# Autodesk Inventor assembly: Mechaniczny_panel_tylny_regal_V1_1
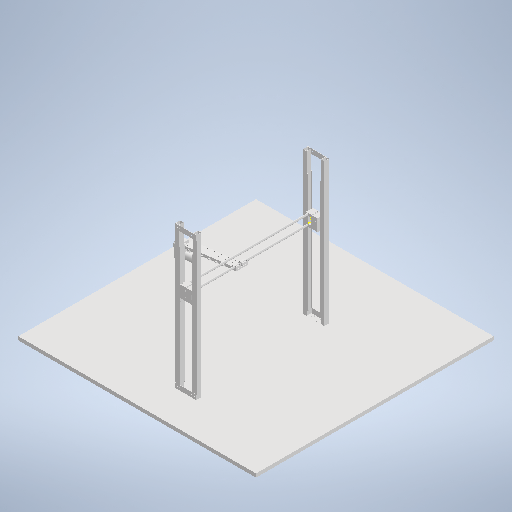
[picture p0: Inventor's stored thumbnail of the model, 512x512]
Saved by Autodesk Inventor 2025.2 (Build 292293000, 293)
## iProperties
Created: 2025-03-18
Part Number: Mechaniczny_panel_tylny_regal_V1_1
Document SubType Name: Assembly
Designer: tadek
Author: tadek
## Documents named in this file (30)
- C:\Users\tadek\Documents\Inventor_projekt_inzynierski\Mechaniczny_panel_tylny_regal_V1_1.iam
- C:\Users\tadek\Documents\Inventor_projekt_inzynierski\lacznik_plaski_180_40_2p5.ipt
- C:\Users\tadek\Documents\Inventor_projekt_inzynierski\podstawa_plyta_200_200_3.ipt
- C:\Users\tadek\Documents\Inventor_projekt_inzynierski\profil_stalowy_40_30_120_MIR.ipt
- C:\Users\tadek\Documents\Inventor_projekt_inzynierski\katownik_lacznikowy_40_40_40.ipt
- C:\Users\tadek\Documents\Inventor_projekt_inzynierski\prowadnica_profil_c.ipt
- C:\Users\tadek\Documents\Inventor_projekt_inzynierski\prowadnica_profil_c_MIR.ipt
- C:\Users\tadek\Documents\Inventor_projekt_inzynierski\lozysko.ipt
- C:\Users\tadek\Documents\Inventor_projekt_inzynierski\lozysko_MIR.ipt
- C:\Users\tadek\Documents\Inventor_projekt_inzynierski\katownik_lacznikowy_40_40_40_MIR1.ipt
- C:\Users\tadek\Documents\Inventor_projekt_inzynierski\lacznik_lozyskowy.ipt
- C:\Users\tadek\Documents\Inventor\Content Center Files\R2025\pl-PL\PEM Self-Clinching Studs FH4,FHP - Metric\FH4-M5-8.ipt
- C:\Users\tadek\Documents\Inventor_projekt_inzynierski\nakretka.ipt
- C:\Users\tadek\Documents\Inventor_projekt_inzynierski\profil_stalowy_40_30_120_MIR_MIR1.ipt
- C:\Users\tadek\Documents\Inventor_projekt_inzynierski\prowadnica_profil_c_MIR2.ipt
- C:\Users\tadek\Documents\Inventor_projekt_inzynierski\prowadnica_profil_c_MIR_MIR1.ipt
- C:\Users\tadek\Documents\Inventor_projekt_inzynierski\lozysko_MIR2.ipt
- C:\Users\tadek\Documents\Inventor_projekt_inzynierski\lozysko_MIR_MIR1.ipt
- C:\Users\tadek\Documents\Inventor_projekt_inzynierski\lacznik_lozyskowy_MIR.ipt
- C:\Users\tadek\Documents\Inventor_projekt_inzynierski\nakretka_MIR.ipt
- C:\Users\tadek\Documents\Inventor_projekt_inzynierski\Zespół1.iam
- C:\Users\tadek\Documents\Inventor_projekt_inzynierski\profil_stalowy_40_30_120_MIR_MIR1_CPY.ipt
- C:\Users\tadek\Documents\Inventor_projekt_inzynierski\profil_stalowy_40_30_120_MIR_CPY.ipt
- C:\Users\tadek\Documents\Inventor_projekt_inzynierski\katownik_lacznikowy_40_40_40_CPY.ipt
- C:\Users\tadek\Documents\Inventor_projekt_inzynierski\katownik_lacznikowy_40_40_40_MIR1_CPY.ipt
- C:\Users\tadek\Documents\Inventor_projekt_inzynierski\lacznik_plaski_180_40_2p5_CPY.ipt
- C:\Users\tadek\Documents\Inventor_projekt_inzynierski\prowadnica_profil_c_CPY.ipt
- C:\Users\tadek\Documents\Inventor_projekt_inzynierski\prowadnica_profil_c_MIR2_CPY.ipt
- C:\Users\tadek\Documents\Inventor_projekt_inzynierski\prowadnica_profil_c_MIR_CPY.ipt
- C:\Users\tadek\Documents\Inventor_projekt_inzynierski\prowadnica_profil_c_MIR_MIR1_CPY.ipt
## Components (50 placed, 29 different names)
1. Zespół1:1 [sub-assembly] — Zestawiające:103, Zestawiające:104, Zestawiające:109, Zestawiające:110, Zestawiające:112, Zestawiające:113, Zestawiające:114, Zestawiające:115, Zestawiające:116, Zestawiające:119, Zestawiające:120, Zestawiające:121, Zestawiające:195, Zestawiające:223, Zestawiające:225, Zestawiające:226, Zestawiające:227, Zestawiające:228, Zestawiające:242, Zestawiające:243
2. podstawa_plyta_200_200_3:1 — Równoległe:9, Równoległe:11, Zestawiające:22, Zestawiające:39, Zestawiające:40, Zestawiające:41, Zestawiające:42, Zestawiające:43, Zestawiające:91, Zestawiające:92, Zestawiające:187, Zestawiające:188, Zestawiające:191, Zestawiające:192, Zestawiające:193, Zestawiające:194
3. profil_stalowy_40_30_120_MIR_MIR1:1 — Zestawiające:63, Zestawiające:64, Zestawiające:65, Zestawiające:66, Zestawiające:67, Zestawiające:68, Zestawiające:74, Zestawiające:75, Zestawiające:76, Zestawiające:77, Zestawiające:93, Zestawiające:94, Zestawiające:95, Zestawiające:96, Zestawiające:123, Zestawiające:124
4. profil_stalowy_40_30_120_MIR:1 — Równoległe:6, Równoległe:8, Zestawiające:4, Zestawiające:5, Równoległe:9, Zestawiające:7, Zestawiające:9, Zestawiające:10, Zestawiające:11, Zestawiające:12, Zestawiające:13, Zestawiające:14, Zestawiające:15, Zestawiające:20, Zestawiające:21, Zestawiające:44, Zestawiające:45, Zestawiające:46, Zestawiające:47, Zestawiające:122
5. lacznik_lozyskowy:1 — Zestawiające:51, Zestawiające:53, Zestawiające:52, Zestawiające:54, Zestawiające:103, Zestawiające:109, Zestawiające:110, Zestawiające:112, Zestawiające:113
6. lacznik_lozyskowy_MIR:1 — Zestawiające:71, Zestawiające:104, Zestawiające:105, Zestawiające:106, Zestawiające:114, Zestawiające:115, Zestawiające:116, Zestawiające:119, Zestawiające:120, Zestawiające:121
7. katownik_lacznikowy_40_40_40:1 — Zestawiające:7, Równoległe:11, Zestawiające:9, Zestawiające:20, Zestawiające:21, Zestawiające:22, Zestawiające:42, Zestawiające:43, Zestawiające:44, Zestawiające:45, Zestawiające:46
8. katownik_lacznikowy_40_40_40_MIR1:1 — Zestawiające:39, Zestawiające:40, Zestawiające:41, Zestawiające:74, Zestawiające:75, Zestawiające:76, Zestawiające:77, Zestawiające:91, Zestawiające:92
9. lacznik_plaski_180_40_2p5:1 — Zestawiające:4, Zestawiające:5, Zestawiające:95, Zestawiające:96, Zestawiające:122, Zestawiające:123, Zestawiające:124
10. lacznik_plaski_180_40_2p5:2 — Zestawiające:47, Zestawiające:93, Zestawiające:94
11. prowadnica_profil_c:2 — Zestawiające:10, Zestawiające:11, Zestawiające:12, Zestawiające:16, Zestawiające:17
12. prowadnica_profil_c_MIR2:1 — Zestawiające:63, Zestawiające:64, Zestawiające:65, Zestawiające:69
13. prowadnica_profil_c_MIR:1 — Zestawiające:13, Zestawiające:14, Zestawiające:15, Zestawiające:18, Zestawiające:19
14. prowadnica_profil_c_MIR_MIR1:1 — Zestawiające:66, Zestawiające:67, Zestawiające:68, Zestawiające:70, Równoległe:15
15. PEM Śruba dwustronna samozaciskowa FH4,FHP - Metryczny FH4-M5-8:2 — Zestawiające:53, Zestawiające:54, Zestawiające:55, Zestawiające:57, Zestawiające:111
16. PEM Śruba dwustronna samozaciskowa FH4,FHP - Metryczny FH4-M5-8:1 — Zestawiające:51, Zestawiające:52, Zestawiające:56, Zestawiające:59
17. PEM Śruba dwustronna samozaciskowa FH4,FHP - Metryczny FH4-M5-8:3 — Zestawiające:86, Zestawiające:90, Zestawiające:105, Zestawiające:118
18. PEM Śruba dwustronna samozaciskowa FH4,FHP - Metryczny FH4-M5-8:4 — Zestawiające:85, Zestawiające:89, Zestawiające:106, Zestawiające:117
19. nakretka:1 — Zestawiające:59, Zestawiające:62
20. nakretka_MIR:1 — Zestawiające:72, Zestawiające:89, Zestawiające:117
21. nakretka:2 — Zestawiające:57, Zestawiające:61, Zestawiające:111
22. nakretka_MIR:2 — Zestawiające:73, Zestawiające:90, Zestawiające:118
23. lozysko:1 — Zestawiające:16, Zestawiające:17, Zestawiające:56, Zestawiające:62
24. lozysko_MIR:1 — Zestawiające:18, Zestawiające:19, Zestawiające:55, Zestawiające:61
25. lozysko_MIR2:1 — Zestawiające:69, Zestawiające:71, Zestawiające:72, Zestawiające:85
26. lozysko_MIR_MIR1:1 — Zestawiające:70, Równoległe:15, Zestawiające:73, Zestawiające:86
27. profil_stalowy_40_30_120_MIR_CPY:1 — Zestawiające:125, Zestawiające:126, Zestawiające:127, Równoległe:17, Zestawiające:128, Zestawiające:129, Zestawiające:130, Zestawiające:131, Zestawiające:132, Zestawiające:133, Zestawiające:134, Zestawiające:135, Zestawiające:136, Zestawiające:137, Zestawiające:138, Zestawiające:139, Zestawiające:140, Zestawiające:145, Równoległe:19
28. profil_stalowy_40_30_120_MIR_MIR1_CPY:1 — Zestawiające:157, Zestawiające:158, Zestawiające:159, Zestawiające:160, Zestawiające:161, Zestawiające:162, Zestawiające:163, Zestawiające:164, Zestawiające:165, Zestawiające:166, Zestawiające:167, Zestawiające:168, Zestawiające:169, Zestawiające:170, Zestawiające:171, Zestawiające:172
29. lacznik_lozyskowy:2 — Zestawiające:242, Zestawiające:243
30. lacznik_lozyskowy_MIR:2 — Zestawiające:222, Zestawiające:223, Zestawiające:225, Zestawiające:226, Zestawiające:227, Zestawiające:228
31. lacznik_plaski_180_40_2p5_CPY:2 — Zestawiające:145, Zestawiające:161, Zestawiające:162
32. lacznik_plaski_180_40_2p5_CPY:1 — Zestawiające:125, Zestawiające:126, Zestawiające:127, Zestawiające:157, Zestawiające:158, Zestawiające:159, Zestawiające:160
33. katownik_lacznikowy_40_40_40_MIR1_CPY:1 — Zestawiające:163, Zestawiające:164, Zestawiające:165, Zestawiające:166, Zestawiające:188, Zestawiające:192, Zestawiające:193, Zestawiające:194
34. katownik_lacznikowy_40_40_40_CPY:1 — Zestawiające:128, Zestawiające:129, Zestawiające:130, Zestawiające:131, Zestawiające:132, Zestawiające:133, Zestawiające:134, Zestawiające:187, Zestawiające:191
35. prowadnica_profil_c_MIR_MIR1_CPY:1 — Zestawiające:170, Zestawiające:171, Zestawiające:172, Zestawiające:245
36. prowadnica_profil_c_MIR_CPY:1 — Zestawiające:138, Zestawiające:139, Zestawiające:140
37. prowadnica_profil_c_MIR2_CPY:1 — Zestawiające:167, Zestawiające:168, Zestawiające:169
38. prowadnica_profil_c_CPY:1 — Zestawiające:135, Zestawiające:136, Zestawiające:137, Zestawiające:244
39. PEM Śruba dwustronna samozaciskowa FH4,FHP - Metryczny FH4-M5-8:12
40. PEM Śruba dwustronna samozaciskowa FH4,FHP - Metryczny FH4-M5-8:11 — Zestawiające:240, Zestawiające:241
41. PEM Śruba dwustronna samozaciskowa FH4,FHP - Metryczny FH4-M5-8:10
42. PEM Śruba dwustronna samozaciskowa FH4,FHP - Metryczny FH4-M5-8:9 — Zestawiające:222
43. nakretka:4
44. nakretka:3 — Zestawiające:241
45. nakretka_MIR:4
46. nakretka_MIR:3
47. lozysko:2 — Zestawiające:240, Zestawiające:245
48. lozysko_MIR:2
49. lozysko_MIR_MIR1:2 — Zestawiające:244
50. lozysko_MIR2:2
## Relationships (162: Mate 155, Flush 7)
- Równoległe:6 [Flush]: profil_stalowy_40_30_120_MIR:1
- Równoległe:8 [Flush] (120 mm): profil_stalowy_40_30_120_MIR:1
- Zestawiające:4 [Mate]: profil_stalowy_40_30_120_MIR:1 ↔ lacznik_plaski_180_40_2p5:1
- Zestawiające:5 [Mate]: profil_stalowy_40_30_120_MIR:1 ↔ lacznik_plaski_180_40_2p5:1
- Równoległe:9 [Flush]: podstawa_plyta_200_200_3:1 ↔ profil_stalowy_40_30_120_MIR:1
- Zestawiające:7 [Mate]: profil_stalowy_40_30_120_MIR:1 ↔ katownik_lacznikowy_40_40_40:1
- Równoległe:11 [Flush]: podstawa_plyta_200_200_3:1 ↔ katownik_lacznikowy_40_40_40:1
- Zestawiające:9 [Mate]: profil_stalowy_40_30_120_MIR:1 ↔ katownik_lacznikowy_40_40_40:1
- Zestawiające:10 [Mate]: profil_stalowy_40_30_120_MIR:1 ↔ prowadnica_profil_c:2
- Zestawiające:11 [Mate]: profil_stalowy_40_30_120_MIR:1 ↔ prowadnica_profil_c:2
- Zestawiające:12 [Mate]: profil_stalowy_40_30_120_MIR:1 ↔ prowadnica_profil_c:2
- Zestawiające:13 [Mate]: profil_stalowy_40_30_120_MIR:1 ↔ prowadnica_profil_c_MIR:1
- Zestawiające:14 [Mate]: profil_stalowy_40_30_120_MIR:1 ↔ prowadnica_profil_c_MIR:1
- Zestawiające:15 [Mate]: profil_stalowy_40_30_120_MIR:1 ↔ prowadnica_profil_c_MIR:1
- Zestawiające:16 [Mate]: prowadnica_profil_c:2 ↔ lozysko:1
- Zestawiające:17 [Mate] (8 mm): prowadnica_profil_c:2 ↔ lozysko:1
- Zestawiające:18 [Mate]: prowadnica_profil_c_MIR:1 ↔ lozysko_MIR:1
- Zestawiające:19 [Mate] (8 mm): prowadnica_profil_c_MIR:1 ↔ lozysko_MIR:1
- Zestawiające:20 [Mate]: profil_stalowy_40_30_120_MIR:1 ↔ katownik_lacznikowy_40_40_40:1
- Zestawiające:21 [Mate]: profil_stalowy_40_30_120_MIR:1 ↔ katownik_lacznikowy_40_40_40:1
- Zestawiające:22 [Mate]: podstawa_plyta_200_200_3:1 ↔ katownik_lacznikowy_40_40_40:1
- Zestawiające:39 [Mate]: podstawa_plyta_200_200_3:1 ↔ katownik_lacznikowy_40_40_40_MIR1:1
- Zestawiające:40 [Mate]: podstawa_plyta_200_200_3:1 ↔ katownik_lacznikowy_40_40_40_MIR1:1
- Zestawiające:41 [Mate]: podstawa_plyta_200_200_3:1 ↔ katownik_lacznikowy_40_40_40_MIR1:1
- Zestawiające:42 [Mate]: podstawa_plyta_200_200_3:1 ↔ katownik_lacznikowy_40_40_40:1
- Zestawiające:43 [Mate]: podstawa_plyta_200_200_3:1 ↔ katownik_lacznikowy_40_40_40:1
- Zestawiające:44 [Mate]: profil_stalowy_40_30_120_MIR:1 ↔ katownik_lacznikowy_40_40_40:1
- Zestawiające:45 [Mate]: profil_stalowy_40_30_120_MIR:1 ↔ katownik_lacznikowy_40_40_40:1
- Zestawiające:46 [Mate]: profil_stalowy_40_30_120_MIR:1 ↔ katownik_lacznikowy_40_40_40:1
- Zestawiające:47 [Mate]: profil_stalowy_40_30_120_MIR:1 ↔ lacznik_plaski_180_40_2p5:2
- Zestawiające:51 [Mate]: lacznik_lozyskowy:1 ↔ PEM Śruba dwustronna samozaciskowa FH4,FHP - Metryczny FH4-M5-8:1
- Zestawiające:53 [Mate]: lacznik_lozyskowy:1 ↔ PEM Śruba dwustronna samozaciskowa FH4,FHP - Metryczny FH4-M5-8:2
- Zestawiające:52 [Mate]: lacznik_lozyskowy:1 ↔ PEM Śruba dwustronna samozaciskowa FH4,FHP - Metryczny FH4-M5-8:1
- Zestawiające:54 [Mate]: lacznik_lozyskowy:1 ↔ PEM Śruba dwustronna samozaciskowa FH4,FHP - Metryczny FH4-M5-8:2
- Zestawiające:55 [Mate]: PEM Śruba dwustronna samozaciskowa FH4,FHP - Metryczny FH4-M5-8:2 ↔ lozysko_MIR:1
- Zestawiające:56 [Mate]: PEM Śruba dwustronna samozaciskowa FH4,FHP - Metryczny FH4-M5-8:1 ↔ lozysko:1
- Zestawiające:57 [Mate]: PEM Śruba dwustronna samozaciskowa FH4,FHP - Metryczny FH4-M5-8:2 ↔ nakretka:2
- Zestawiające:59 [Mate]: PEM Śruba dwustronna samozaciskowa FH4,FHP - Metryczny FH4-M5-8:1 ↔ nakretka:1
- Zestawiające:61 [Mate]: nakretka:2 ↔ lozysko_MIR:1
- Zestawiające:62 [Mate]: nakretka:1 ↔ lozysko:1
- Zestawiające:63 [Mate]: profil_stalowy_40_30_120_MIR_MIR1:1 ↔ prowadnica_profil_c_MIR2:1
- Zestawiające:64 [Mate]: profil_stalowy_40_30_120_MIR_MIR1:1 ↔ prowadnica_profil_c_MIR2:1
- Zestawiające:65 [Mate]: profil_stalowy_40_30_120_MIR_MIR1:1 ↔ prowadnica_profil_c_MIR2:1
- Zestawiające:66 [Mate]: profil_stalowy_40_30_120_MIR_MIR1:1 ↔ prowadnica_profil_c_MIR_MIR1:1
- Zestawiające:67 [Mate]: profil_stalowy_40_30_120_MIR_MIR1:1 ↔ prowadnica_profil_c_MIR_MIR1:1
- Zestawiające:68 [Mate]: profil_stalowy_40_30_120_MIR_MIR1:1 ↔ prowadnica_profil_c_MIR_MIR1:1
- Zestawiające:69 [Mate] (8 mm): prowadnica_profil_c_MIR2:1 ↔ lozysko_MIR2:1
- Zestawiające:70 [Mate] (8 mm): prowadnica_profil_c_MIR_MIR1:1 ↔ lozysko_MIR_MIR1:1
- Równoległe:15 [Flush]: prowadnica_profil_c_MIR_MIR1:1 ↔ lozysko_MIR_MIR1:1
- Zestawiające:71 [Mate]: lacznik_lozyskowy_MIR:1 ↔ lozysko_MIR2:1
- Zestawiające:72 [Mate]: nakretka_MIR:1 ↔ lozysko_MIR2:1
- Zestawiające:73 [Mate]: nakretka_MIR:2 ↔ lozysko_MIR_MIR1:1
- Zestawiające:74 [Mate]: profil_stalowy_40_30_120_MIR_MIR1:1 ↔ katownik_lacznikowy_40_40_40_MIR1:1
- Zestawiające:75 [Mate]: profil_stalowy_40_30_120_MIR_MIR1:1 ↔ katownik_lacznikowy_40_40_40_MIR1:1
- Zestawiające:76 [Mate]: profil_stalowy_40_30_120_MIR_MIR1:1 ↔ katownik_lacznikowy_40_40_40_MIR1:1
- Zestawiające:77 [Mate]: profil_stalowy_40_30_120_MIR_MIR1:1 ↔ katownik_lacznikowy_40_40_40_MIR1:1
- Zestawiające:85 [Mate]: PEM Śruba dwustronna samozaciskowa FH4,FHP - Metryczny FH4-M5-8:4 ↔ lozysko_MIR2:1
- Zestawiające:86 [Mate]: PEM Śruba dwustronna samozaciskowa FH4,FHP - Metryczny FH4-M5-8:3 ↔ lozysko_MIR_MIR1:1
- Zestawiające:89 [Mate]: PEM Śruba dwustronna samozaciskowa FH4,FHP - Metryczny FH4-M5-8:4 ↔ nakretka_MIR:1
- Zestawiające:90 [Mate]: PEM Śruba dwustronna samozaciskowa FH4,FHP - Metryczny FH4-M5-8:3 ↔ nakretka_MIR:2
- Zestawiające:91 [Mate]: podstawa_plyta_200_200_3:1 ↔ katownik_lacznikowy_40_40_40_MIR1:1
- Zestawiające:92 [Mate]: podstawa_plyta_200_200_3:1 ↔ katownik_lacznikowy_40_40_40_MIR1:1
- Zestawiające:93 [Mate]: profil_stalowy_40_30_120_MIR_MIR1:1 ↔ lacznik_plaski_180_40_2p5:2
- Zestawiające:94 [Mate]: profil_stalowy_40_30_120_MIR_MIR1:1 ↔ lacznik_plaski_180_40_2p5:2
- Zestawiające:95 [Mate]: profil_stalowy_40_30_120_MIR_MIR1:1 ↔ lacznik_plaski_180_40_2p5:1
- Zestawiające:96 [Mate]: profil_stalowy_40_30_120_MIR_MIR1:1 ↔ lacznik_plaski_180_40_2p5:1
- Zestawiające:103 [Mate]: Zespół1:1 ↔ lacznik_lozyskowy:1
- Zestawiające:104 [Mate]: Zespół1:1 ↔ lacznik_lozyskowy_MIR:1
- Zestawiające:105 [Mate]: lacznik_lozyskowy_MIR:1 ↔ PEM Śruba dwustronna samozaciskowa FH4,FHP - Metryczny FH4-M5-8:3
- Zestawiające:106 [Mate]: lacznik_lozyskowy_MIR:1 ↔ PEM Śruba dwustronna samozaciskowa FH4,FHP - Metryczny FH4-M5-8:4
- Zestawiające:109 [Mate]: Zespół1:1 ↔ lacznik_lozyskowy:1
- Zestawiające:110 [Mate]: Zespół1:1 ↔ lacznik_lozyskowy:1
- Zestawiające:111 [Mate]: PEM Śruba dwustronna samozaciskowa FH4,FHP - Metryczny FH4-M5-8:2 ↔ nakretka:2
- Zestawiające:112 [Mate]: Zespół1:1 ↔ lacznik_lozyskowy:1
- Zestawiające:113 [Mate]: Zespół1:1 ↔ lacznik_lozyskowy:1
- Zestawiające:114 [Mate]: Zespół1:1 ↔ lacznik_lozyskowy_MIR:1
- Zestawiające:115 [Mate]: Zespół1:1 ↔ lacznik_lozyskowy_MIR:1
- Zestawiające:116 [Mate]: Zespół1:1 ↔ lacznik_lozyskowy_MIR:1
- Zestawiające:117 [Mate]: PEM Śruba dwustronna samozaciskowa FH4,FHP - Metryczny FH4-M5-8:4 ↔ nakretka_MIR:1
- Zestawiające:118 [Mate]: PEM Śruba dwustronna samozaciskowa FH4,FHP - Metryczny FH4-M5-8:3 ↔ nakretka_MIR:2
- Zestawiające:119 [Mate]: Zespół1:1 ↔ lacznik_lozyskowy_MIR:1
- Zestawiające:120 [Mate]: Zespół1:1 ↔ lacznik_lozyskowy_MIR:1
- Zestawiające:121 [Mate]: Zespół1:1 ↔ lacznik_lozyskowy_MIR:1
- Zestawiające:122 [Mate]: profil_stalowy_40_30_120_MIR:1 ↔ lacznik_plaski_180_40_2p5:1
- Zestawiające:123 [Mate]: profil_stalowy_40_30_120_MIR_MIR1:1 ↔ lacznik_plaski_180_40_2p5:1
- Zestawiające:124 [Mate]: profil_stalowy_40_30_120_MIR_MIR1:1 ↔ lacznik_plaski_180_40_2p5:1
- Zestawiające:125 [Mate]: profil_stalowy_40_30_120_MIR_CPY:1 ↔ lacznik_plaski_180_40_2p5_CPY:1
- Zestawiające:126 [Mate]: profil_stalowy_40_30_120_MIR_CPY:1 ↔ lacznik_plaski_180_40_2p5_CPY:1
- Zestawiające:127 [Mate]: profil_stalowy_40_30_120_MIR_CPY:1 ↔ lacznik_plaski_180_40_2p5_CPY:1
- Równoległe:17 [Flush] (120 mm): profil_stalowy_40_30_120_MIR_CPY:1
- Zestawiające:128 [Mate]: profil_stalowy_40_30_120_MIR_CPY:1 ↔ katownik_lacznikowy_40_40_40_CPY:1
- Zestawiające:129 [Mate]: profil_stalowy_40_30_120_MIR_CPY:1 ↔ katownik_lacznikowy_40_40_40_CPY:1
- Zestawiające:130 [Mate]: profil_stalowy_40_30_120_MIR_CPY:1 ↔ katownik_lacznikowy_40_40_40_CPY:1
- Zestawiające:131 [Mate]: profil_stalowy_40_30_120_MIR_CPY:1 ↔ katownik_lacznikowy_40_40_40_CPY:1
- Zestawiające:132 [Mate]: profil_stalowy_40_30_120_MIR_CPY:1 ↔ katownik_lacznikowy_40_40_40_CPY:1
- Zestawiające:133 [Mate]: profil_stalowy_40_30_120_MIR_CPY:1 ↔ katownik_lacznikowy_40_40_40_CPY:1
- Zestawiające:134 [Mate]: profil_stalowy_40_30_120_MIR_CPY:1 ↔ katownik_lacznikowy_40_40_40_CPY:1
- Zestawiające:135 [Mate]: profil_stalowy_40_30_120_MIR_CPY:1 ↔ prowadnica_profil_c_CPY:1
- Zestawiające:136 [Mate]: profil_stalowy_40_30_120_MIR_CPY:1 ↔ prowadnica_profil_c_CPY:1
- Zestawiające:137 [Mate]: profil_stalowy_40_30_120_MIR_CPY:1 ↔ prowadnica_profil_c_CPY:1
- Zestawiające:138 [Mate]: profil_stalowy_40_30_120_MIR_CPY:1 ↔ prowadnica_profil_c_MIR_CPY:1
- Zestawiające:139 [Mate]: profil_stalowy_40_30_120_MIR_CPY:1 ↔ prowadnica_profil_c_MIR_CPY:1
- Zestawiające:140 [Mate]: profil_stalowy_40_30_120_MIR_CPY:1 ↔ prowadnica_profil_c_MIR_CPY:1
- Zestawiające:145 [Mate]: profil_stalowy_40_30_120_MIR_CPY:1 ↔ lacznik_plaski_180_40_2p5_CPY:2
- Zestawiające:157 [Mate]: profil_stalowy_40_30_120_MIR_MIR1_CPY:1 ↔ lacznik_plaski_180_40_2p5_CPY:1
- Zestawiające:158 [Mate]: profil_stalowy_40_30_120_MIR_MIR1_CPY:1 ↔ lacznik_plaski_180_40_2p5_CPY:1
- Zestawiające:159 [Mate]: profil_stalowy_40_30_120_MIR_MIR1_CPY:1 ↔ lacznik_plaski_180_40_2p5_CPY:1
- Zestawiające:160 [Mate]: profil_stalowy_40_30_120_MIR_MIR1_CPY:1 ↔ lacznik_plaski_180_40_2p5_CPY:1
- Zestawiające:161 [Mate]: profil_stalowy_40_30_120_MIR_MIR1_CPY:1 ↔ lacznik_plaski_180_40_2p5_CPY:2
- Zestawiające:162 [Mate]: profil_stalowy_40_30_120_MIR_MIR1_CPY:1 ↔ lacznik_plaski_180_40_2p5_CPY:2
- Zestawiające:163 [Mate]: profil_stalowy_40_30_120_MIR_MIR1_CPY:1 ↔ katownik_lacznikowy_40_40_40_MIR1_CPY:1
- Zestawiające:164 [Mate]: profil_stalowy_40_30_120_MIR_MIR1_CPY:1 ↔ katownik_lacznikowy_40_40_40_MIR1_CPY:1
- Zestawiające:165 [Mate]: profil_stalowy_40_30_120_MIR_MIR1_CPY:1 ↔ katownik_lacznikowy_40_40_40_MIR1_CPY:1
- Zestawiające:166 [Mate]: profil_stalowy_40_30_120_MIR_MIR1_CPY:1 ↔ katownik_lacznikowy_40_40_40_MIR1_CPY:1
- Zestawiające:167 [Mate]: profil_stalowy_40_30_120_MIR_MIR1_CPY:1 ↔ prowadnica_profil_c_MIR2_CPY:1
- Zestawiające:168 [Mate]: profil_stalowy_40_30_120_MIR_MIR1_CPY:1 ↔ prowadnica_profil_c_MIR2_CPY:1
- Zestawiające:169 [Mate]: profil_stalowy_40_30_120_MIR_MIR1_CPY:1 ↔ prowadnica_profil_c_MIR2_CPY:1
- Zestawiające:170 [Mate]: profil_stalowy_40_30_120_MIR_MIR1_CPY:1 ↔ prowadnica_profil_c_MIR_MIR1_CPY:1
- Zestawiające:171 [Mate]: profil_stalowy_40_30_120_MIR_MIR1_CPY:1 ↔ prowadnica_profil_c_MIR_MIR1_CPY:1
- Zestawiające:172 [Mate]: profil_stalowy_40_30_120_MIR_MIR1_CPY:1 ↔ prowadnica_profil_c_MIR_MIR1_CPY:1
- Zestawiające:187 [Mate]: podstawa_plyta_200_200_3:1 ↔ katownik_lacznikowy_40_40_40_CPY:1
- Zestawiające:188 [Mate]: podstawa_plyta_200_200_3:1 ↔ katownik_lacznikowy_40_40_40_MIR1_CPY:1
- Zestawiające:191 [Mate]: podstawa_plyta_200_200_3:1 ↔ katownik_lacznikowy_40_40_40_CPY:1
- Zestawiające:192 [Mate]: podstawa_plyta_200_200_3:1 ↔ katownik_lacznikowy_40_40_40_MIR1_CPY:1
- Zestawiające:193 [Mate]: podstawa_plyta_200_200_3:1 ↔ katownik_lacznikowy_40_40_40_MIR1_CPY:1
- Zestawiające:194 [Mate]: podstawa_plyta_200_200_3:1 ↔ katownik_lacznikowy_40_40_40_MIR1_CPY:1
- Równoległe:19 [Flush] (-38 mm): profil_stalowy_40_30_120_MIR_CPY:1
- Zestawiające:195 [Mate]: Zespół1:1
- [Mate]: lacznik_lozyskowy_MIR:2 ↔ lozysko_MIR2:2
- [Mate]: nakretka_MIR:3 ↔ lozysko_MIR2:2
- [Mate]: nakretka_MIR:4 ↔ lozysko_MIR_MIR1:2
- [Mate]: PEM Śruba dwustronna samozaciskowa FH4,FHP - Metryczny FH4-M5-8:10 ↔ lozysko_MIR2:2
- [Mate]: PEM Śruba dwustronna samozaciskowa FH4,FHP - Metryczny FH4-M5-8:9 ↔ lozysko_MIR_MIR1:2
- [Mate]: PEM Śruba dwustronna samozaciskowa FH4,FHP - Metryczny FH4-M5-8:10 ↔ nakretka_MIR:3
- [Mate]: PEM Śruba dwustronna samozaciskowa FH4,FHP - Metryczny FH4-M5-8:9 ↔ nakretka_MIR:4
- [Mate]: lacznik_lozyskowy_MIR:2 ↔ PEM Śruba dwustronna samozaciskowa FH4,FHP - Metryczny FH4-M5-8:9
- [Mate]: lacznik_lozyskowy_MIR:2 ↔ PEM Śruba dwustronna samozaciskowa FH4,FHP - Metryczny FH4-M5-8:10
- [Mate]: PEM Śruba dwustronna samozaciskowa FH4,FHP - Metryczny FH4-M5-8:10 ↔ nakretka_MIR:3
- [Mate]: PEM Śruba dwustronna samozaciskowa FH4,FHP - Metryczny FH4-M5-8:9 ↔ nakretka_MIR:4
- Zestawiające:222 [Mate]: lacznik_lozyskowy_MIR:2 ↔ PEM Śruba dwustronna samozaciskowa FH4,FHP - Metryczny FH4-M5-8:9
- Zestawiające:223 [Mate]: Zespół1:1 ↔ lacznik_lozyskowy_MIR:2
- Zestawiające:225 [Mate]: Zespół1:1 ↔ lacznik_lozyskowy_MIR:2
- Zestawiające:226 [Mate]: Zespół1:1 ↔ lacznik_lozyskowy_MIR:2
- Zestawiające:227 [Mate]: Zespół1:1 ↔ lacznik_lozyskowy_MIR:2
- Zestawiające:228 [Mate]: Zespół1:1 ↔ lacznik_lozyskowy_MIR:2
- [Mate]: lacznik_lozyskowy:2 ↔ PEM Śruba dwustronna samozaciskowa FH4,FHP - Metryczny FH4-M5-8:11
- [Mate]: lacznik_lozyskowy:2 ↔ PEM Śruba dwustronna samozaciskowa FH4,FHP - Metryczny FH4-M5-8:12
- [Mate]: lacznik_lozyskowy:2 ↔ PEM Śruba dwustronna samozaciskowa FH4,FHP - Metryczny FH4-M5-8:11
- [Mate]: lacznik_lozyskowy:2 ↔ PEM Śruba dwustronna samozaciskowa FH4,FHP - Metryczny FH4-M5-8:12
- [Mate]: PEM Śruba dwustronna samozaciskowa FH4,FHP - Metryczny FH4-M5-8:12 ↔ lozysko_MIR:2
- [Mate]: PEM Śruba dwustronna samozaciskowa FH4,FHP - Metryczny FH4-M5-8:11 ↔ lozysko:2
- [Mate]: PEM Śruba dwustronna samozaciskowa FH4,FHP - Metryczny FH4-M5-8:12 ↔ nakretka:4
- [Mate]: PEM Śruba dwustronna samozaciskowa FH4,FHP - Metryczny FH4-M5-8:11 ↔ nakretka:3
- [Mate]: nakretka:4 ↔ lozysko_MIR:2
- [Mate]: nakretka:3 ↔ lozysko:2
- [Mate]: PEM Śruba dwustronna samozaciskowa FH4,FHP - Metryczny FH4-M5-8:12 ↔ nakretka:4
- Zestawiające:240 [Mate]: PEM Śruba dwustronna samozaciskowa FH4,FHP - Metryczny FH4-M5-8:11 ↔ lozysko:2
- Zestawiające:241 [Mate]: PEM Śruba dwustronna samozaciskowa FH4,FHP - Metryczny FH4-M5-8:11 ↔ nakretka:3
- Zestawiające:242 [Mate]: Zespół1:1 ↔ lacznik_lozyskowy:2
- Zestawiające:243 [Mate]: Zespół1:1 ↔ lacznik_lozyskowy:2
- Zestawiające:244 [Mate]: prowadnica_profil_c_CPY:1 ↔ lozysko_MIR_MIR1:2
- Zestawiające:245 [Mate]: prowadnica_profil_c_MIR_MIR1_CPY:1 ↔ lozysko:2
## Named parameters: d303_d111 = 0 mm, d304_d112 = 0 mm, d305_d113 = 0 mm, d306_d125 = 0 mm, d307_d126 = 0 mm, d308_d129 = 0 mm, d309_d130 = 0 mm, d310_d188 = 0 mm, d311_d189 = 0 mm, d312_d176 = 0 mm, d313_d177 = 0 mm, d321_d86 = 0 mm, d322_d87 = 0 mm, d323_d88 = 0 mm, d324_d89 = 0 mm, d325_d90 = 0 mm, d326_d91 = 0 mm, d327_d92 = 0 mm, d328_d94 = 0 mm, d329_d97 = 0 mm, d330_d98 = 0 mm, d331_d182 = 0 mm
